# Autodesk Inventor assembly: robot_top
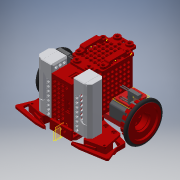
[picture p0: Inventor's stored thumbnail of the model, 180x180]
Saved by Autodesk Inventor 2016 (Build 200138000, 138)
## iProperties
Created: 2016-02-13
Part Number: robot_top
Document SubType Name: Assembly
Designer: jforce
Author: jforce
## Documents named in this file (10)
- C:\Users\jforce\Dropbox\gmu\ece590\robot_models\robot_top.iam
- C:\Users\jforce\Dropbox\gmu\ece590\robot_models\chassis_plate.ipt
- C:\Users\jforce\Dropbox\gmu\ece590\robot_models\robotis_pi_box.iam
- C:\Users\jforce\Dropbox\gmu\ece590\robot_models\r_wheel_assembly.iam
- C:\Users\jforce\Dropbox\gmu\ece590\robot_models\l_wheel_assembly.iam
- C:\Users\jforce\Dropbox\gmu\ece590\robot_models\opencm9_grp.iam
- C:\Users\jforce\Dropbox\gmu\ece590\robot_models\batt.iam
- C:\Users\jforce\Dropbox\gmu\ece590\robot_models\batt_MIR1.iam
- C:\Users\jforce\Dropbox\gmu\ece590\robot_models\bumper.iam
- C:\Users\jforce\Dropbox\gmu\ece590\robot_models\caster_pad.ipt
## Components (9 placed, 9 different names)
1. chassis_plate:1 — Mate:23, Mate:24, Mate:25, Mate:26, Mate:27, Mate:28, Mate:29, Mate:30, Mate:32
2. robotis_pi_box:1 [sub-assembly] — Mate:29, Mate:31, Mate:32, Mate:34, Mate:35, Mate:36, Mate:37, Mate:38, Angle:1, Symmetry:1
3. r_wheel_assembly:1 [sub-assembly] — Mate:26, Mate:27, Mate:28
4. l_wheel_assembly:1 [sub-assembly] — Mate:23, Mate:24, Mate:25, Mate:30
5. opencm9_grp:1 [sub-assembly] — Mate:31, Mate:37
6. batt:2 [sub-assembly] — Mate:34, Mate:35, Mate:36
7. batt_MIR1:1 [sub-assembly]
8. bumper:1 [sub-assembly] — Mate:39, Angle:2, Mate:40, Mate:41, Mate:42, Mate:43
9. caster_pad:1 — Mate:40, Mate:41, Mate:42, Mate:43
## Relationships (23: Mate 20, Angle 2, Symmetry 1)
- Mate:23: chassis_plate:1 ↔ l_wheel_assembly:1
- Mate:24: chassis_plate:1 ↔ l_wheel_assembly:1
- Mate:25: chassis_plate:1 ↔ l_wheel_assembly:1
- Mate:26: chassis_plate:1 ↔ r_wheel_assembly:1
- Mate:27: chassis_plate:1 ↔ r_wheel_assembly:1
- Mate:28: chassis_plate:1 ↔ r_wheel_assembly:1
- Mate:29: chassis_plate:1 ↔ robotis_pi_box:1
- Mate:30: chassis_plate:1 ↔ l_wheel_assembly:1
- Mate:31: robotis_pi_box:1 ↔ opencm9_grp:1
- Mate:32: chassis_plate:1 ↔ robotis_pi_box:1
- Mate:34: robotis_pi_box:1 ↔ batt:2
- Mate:35: robotis_pi_box:1 ↔ batt:2
- Mate:36: robotis_pi_box:1 ↔ batt:2
- Mate:37: robotis_pi_box:1 ↔ opencm9_grp:1
- Mate:38: robotis_pi_box:1
- Angle:1 (0 deg): robotis_pi_box:1
- Symmetry:1: robotis_pi_box:1
- Mate:39: bumper:1
- Angle:2 (0 deg): bumper:1
- Mate:40: bumper:1 ↔ caster_pad:1
- Mate:41: bumper:1 ↔ caster_pad:1
- Mate:42: bumper:1 ↔ caster_pad:1
- Mate:43: bumper:1 ↔ caster_pad:1
